# Autodesk Inventor assembly: Roller Assembly
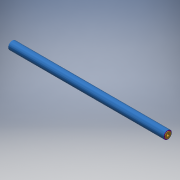
[picture p0: Inventor's stored thumbnail of the model, 180x180]
Saved by Autodesk Inventor 2017 (Build 210142000, 142)
## iProperties
Created: 2017-01-14
Part Number: Roller Assembly
Document SubType Name: Assembly
Designer: Ben
Author: Ben
## Documents named in this file (3)
- C:\Users\Ben\Desktop\Projects\2017 Robot\Ball Intake\Roller Assembly.iam
- C:\Users\Ben\Desktop\Projects\2017 Robot\Ball Intake\1in PVC Roller.ipt
- C:\Users\Ben\Desktop\Projects\2017 Robot\Ball Intake\Roller End Plug.ipt
## Components (3 placed, 2 different names)
1. 1in PVC Roller:1 — Insert:1, Insert:2
2. Roller End Plug:1 — Insert:1
3. Roller End Plug:2 — Insert:2
## Relationships (2: Insert 2)
- Insert:1: 1in PVC Roller:1 ↔ Roller End Plug:1
- Insert:2: 1in PVC Roller:1 ↔ Roller End Plug:2
